# Autodesk Inventor assembly: Assembly - armCentered
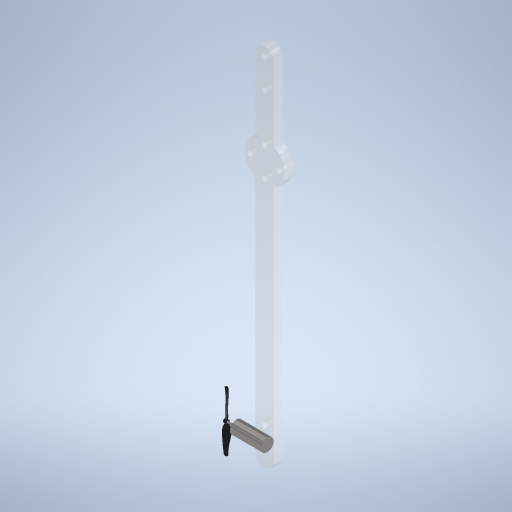
[picture p0: Inventor's stored thumbnail of the model, 512x512]
Saved by Autodesk Inventor 2023.1 (Build 271208000, 208)
## iProperties
Created: 2023-05-09
Part Number: Assembly - armCentered
Document SubType Name: Assembly
Designer: felip
Author: felip
## Documents named in this file (4)
- C:\Users\felip\OneDrive\UNAL FORE\SEMESTRE 9\TECNICAS DE CONTROL\PROYECTO\PROYECTO-TDC-INVENTOR\Assembly - armCentered.iam
- C:\Users\felip\OneDrive\UNAL FORE\SEMESTRE 9\TECNICAS DE CONTROL\PROYECTO\PROYECTO-TDC-INVENTOR\brazo.ipt
- C:\Users\felip\OneDrive\UNAL FORE\SEMESTRE 9\TECNICAS DE CONTROL\PROYECTO\PROYECTO-TDC-INVENTOR\motor.ipt
- C:\Users\felip\OneDrive\UNAL FORE\SEMESTRE 9\TECNICAS DE CONTROL\PROYECTO\PROYECTO-TDC-INVENTOR\helice.ipt
## Components (3 placed, 3 different names)
1. brazo:1 — Flush:1, Tangent:1, Tangent:2
2. motor:1 — Flush:1, Tangent:1, Angle:1, Mate:1, Rotational:1
3. helice:1 — Rotational:1
## Relationships (6: Tangent 2, Flush 1, Angle 1, Mate 1, RevoluteJoint 1)
- Flush:1: brazo:1 ↔ motor:1
- Tangent:1: brazo:1 ↔ motor:1
- Angle:1 (0 deg): motor:1
- Tangent:2: brazo:1
- Mate:1 (-15.5 mm): motor:1
- Rotational:1 [RevoluteJoint]: motor:1 ↔ helice:1
